# Autodesk Inventor assembly: CorteSección
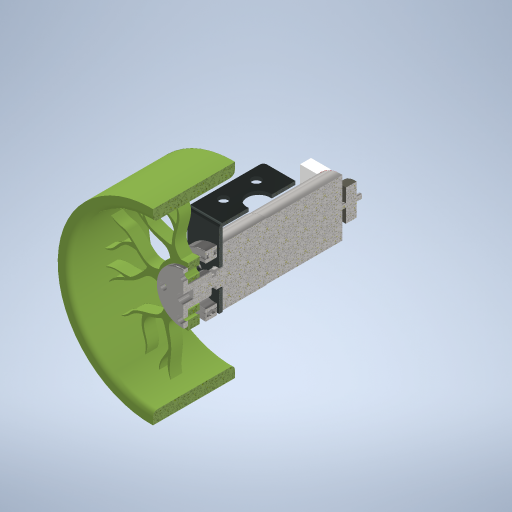
[picture p0: Inventor's stored thumbnail of the model, 512x512]
Saved by Autodesk Inventor 2024.2 (Build 282272000, 272)
## iProperties
Created: 2025-07-17
Part Number: CorteSección
Document SubType Name: Assembly
Designer: Admin
Author: Admin
## Documents named in this file (6)
- C:\Users\Admin\Documents\GitHub\ExplorateurErrant\Assemblies\CorteSección.iam
- C:\Users\Admin\Documents\GitHub\ExplorateurErrant\Motors\DC-JGA25\WH-Bracket-JGA25.ipt
- C:\Users\Admin\Documents\GitHub\ExplorateurErrant\Wheels\RodamientoTest\61803-2rs1.iam
- C:\Users\Admin\Documents\GitHub\ExplorateurErrant\Motors\DC-JGA25\WH-Coupling-4mm.ipt
- C:\Users\Admin\Documents\GitHub\ExplorateurErrant\Wheels\RhymTest.ipt
- C:\Users\Admin\Documents\GitHub\ExplorateurErrant\Motors\DC-JGA25\WH-Motor-JGA25.ipt
## Components (5 placed, 5 different names)
1. WH-Bracket-JGA25:1 — Mate:4, Mate:5, Mate:6, Mate:7, Mate:8
2. 61803-2rs1:1 [sub-assembly] — Mate:4
3. WH-Coupling-4mm:1 — Mate:1, Mate:2, Mate:3, Mate:5
4. RhymTest:1 — Mate:1, Mate:2, Mate:3
5. WH-Motor-JGA25:1 — Mate:6, Mate:7, Mate:8
## Relationships (8: Mate 8)
- Mate:1: WH-Coupling-4mm:1 ↔ RhymTest:1
- Mate:2: WH-Coupling-4mm:1 ↔ RhymTest:1
- Mate:3: WH-Coupling-4mm:1 ↔ RhymTest:1
- Mate:4: WH-Bracket-JGA25:1 ↔ 61803-2rs1:1
- Mate:5: WH-Bracket-JGA25:1 ↔ WH-Coupling-4mm:1
- Mate:6: WH-Bracket-JGA25:1 ↔ WH-Motor-JGA25:1
- Mate:7: WH-Bracket-JGA25:1 ↔ WH-Motor-JGA25:1
- Mate:8: WH-Bracket-JGA25:1 ↔ WH-Motor-JGA25:1
